# Autodesk Inventor assembly: Zlozenie_MD_Drone
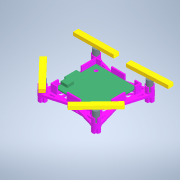
[picture p0: Inventor's stored thumbnail of the model, 180x180]
Saved by Autodesk Inventor 2022 (Build 260153000, 153)
## iProperties
Created: 2021-08-11
Part Number: Zlozenie_MD_Drone
Document SubType Name: Assembly
Designer: Krystyna
Mass: 86 g
Surface Area: 434.756 cm^2
Volume: 46.6468 cm^3
Author: Krystyna
## Documents named in this file (6)
- C:\Users\Krystyna\Documents\MD_V2\Rama\Zlozenie_MD_Drone.iam
- C:\Users\Krystyna\Documents\MD_V2\Rama\Obudowa_dol.ipt
- C:\Users\Krystyna\Documents\MD_V2\Rama\PCB.ipt
- C:\Users\Krystyna\Documents\MD_V2\Rama\Bateria.ipt
- C:\Users\Krystyna\Documents\MD_V2\Rama\Silnik.ipt
- C:\Users\Krystyna\Documents\MD_V2\Rama\Smiglo.ipt
## Components (11 placed, 5 different names)
1. Obudowa_dol:1 — Obrotowe:1, Obrotowe:2, Obrotowe:3, Obrotowe:4, Obrotowe:5, Sztywne:1
2. PCB:1 — Obrotowe:1
3. Bateria:1 — Sztywne:1
4. Silnik:1 — Obrotowe:2, Obrotowe:9
5. Silnik:2 — Obrotowe:3, Obrotowe:7
6. Silnik:3 — Obrotowe:4, Obrotowe:6
7. Silnik:4 — Obrotowe:5, Obrotowe:8
8. Smiglo:1 — Obrotowe:6
9. Smiglo:2 — Obrotowe:7
10. Smiglo:3 — Obrotowe:8
11. Smiglo:4 — Obrotowe:9
## Relationships (10: RevoluteJoint 9, WeldJoint 1)
- Obrotowe:1 [RevoluteJoint]: Obudowa_dol:1 ↔ PCB:1
- Obrotowe:2 [RevoluteJoint]: Obudowa_dol:1 ↔ Silnik:1
- Obrotowe:3 [RevoluteJoint]: Obudowa_dol:1 ↔ Silnik:2
- Obrotowe:4 [RevoluteJoint]: Obudowa_dol:1 ↔ Silnik:3
- Obrotowe:5 [RevoluteJoint]: Obudowa_dol:1 ↔ Silnik:4
- Sztywne:1 [WeldJoint]: Obudowa_dol:1 ↔ Bateria:1
- Obrotowe:6 [RevoluteJoint]: Silnik:3 ↔ Smiglo:1
- Obrotowe:7 [RevoluteJoint]: Silnik:2 ↔ Smiglo:2
- Obrotowe:8 [RevoluteJoint]: Silnik:4 ↔ Smiglo:3
- Obrotowe:9 [RevoluteJoint]: Silnik:1 ↔ Smiglo:4
